# Autodesk Inventor assembly: FrisbeeShooter
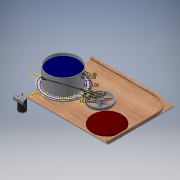
[picture p0: Inventor's stored thumbnail of the model, 180x180]
Saved by Autodesk Inventor 2016 (Build 200138000, 138)
## iProperties
Created: 2015-07-20
Part Number: FrisbeeShooter
Document SubType Name: Assembly
Designer: steele
Mass: 4574.46 g
Surface Area: 17770.7 cm^2
Volume: 6674.99 cm^3
Density: 0.685314 g/cm^3
Author: steele
## Documents named in this file (10)
- C:\snobotics\CAD-Development\robSteele\FRC 2013 Ultimate Ascent\FrisbeeShooter.iam
- C:\snobotics\CAD-Development\robSteele\FRC 2013 Ultimate Ascent\FrisbeeHopper.ipt
- C:\snobotics\ptc\FRC 2013 Ultimate Acsent\FRC_KOP\2013_frc_kop\Black Tote\53214-b_2013.ipt
- C:\snobotics\CAD-Development\robSteele\FRC 2013 Ultimate Ascent\DiskCam.ipt
- C:\snobotics\CAD-Development\robSteele\FRC 2013 Ultimate Ascent\ShooterBase.ipt
- C:\snobotics\CAD-MfgResources\Andy-Mark\Wheels\8 in Diameter\x2010-8-FIRSTwheel-375bear.ipt
- C:\snobotics\CAD-MfgResources\Andy-Mark\Hubs\am-0134a+375+Key+Hub+r2.ipt
- C:\snobotics\CAD-MfgResources\Andy-Mark\MotorMounts\AM 2488 CIM bracket.ipt
- C:\snobotics\autodesk\2015\FRC_KOP_2015\Motors\MOT_CIM-Motor_217-2000.iam
- C:\snobotics\ptc\FRC 2013 Ultimate Acsent\FRC_KOP\2013_frc_kop\Black Tote\53214-r_2013.ipt
## Components (9 placed, 9 different names)
1. ShooterBase:1 — Flush:1
2. FrisbeeHopper:1 — Insert:1, Insert:5
3. 53214-b_2013:1 — Insert:1
4. x2010-8-FIRSTwheel-375bear:1 — Insert:3
5. am-0134a+375+Key+Hub+r2:1 — Insert:3
6. AM 2488 CIM bracket:1 — Insert:4
7. MOT_CIM-Motor_217-2000:1 [sub-assembly] — Insert:4
8. DiskCam:1 — Insert:5
9. 53214-r_2013:1 — Flush:1
## Relationships (5: Insert 4, Flush 1)
- Insert:1: FrisbeeHopper:1 ↔ 53214-b_2013:1
- Insert:3: x2010-8-FIRSTwheel-375bear:1 ↔ am-0134a+375+Key+Hub+r2:1
- Insert:4: AM 2488 CIM bracket:1 ↔ MOT_CIM-Motor_217-2000:1
- Insert:5: FrisbeeHopper:1 ↔ DiskCam:1
- Flush:1 (35.56 mm): ShooterBase:1 ↔ 53214-r_2013:1
